# Autodesk Inventor assembly: Kippschalter
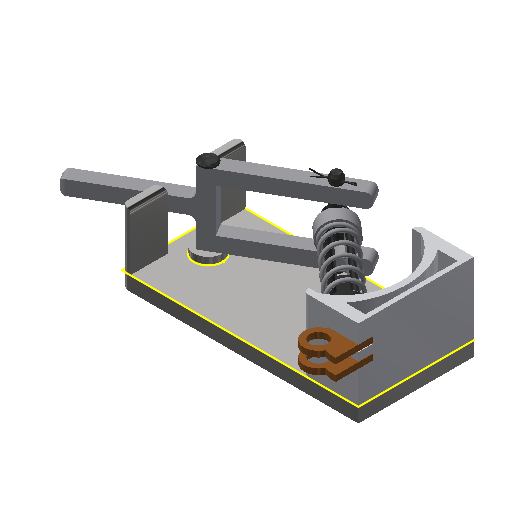
[picture p0: Inventor's stored thumbnail of the model, 512x512]
Saved by Autodesk Inventor 2025.3 (Build 293356000, 356)
## iProperties
Created: 2025-01-24
Part Number: Kippschalter
Material: Generisch
Document SubType Name: Assembly
Designer: abdel
Author: abdel
## Documents named in this file (12)
- C:\Users\abdel\Documents\Inventor\Projektname\Beleg Me2\Kippschalter.iam
- C:\Users\abdel\Documents\Inventor\Projektname\Beleg Me2\Feder.ipt
- C:\Users\abdel\Documents\Inventor\Projektname\Beleg Me2\Federbalken.ipt
- C:\Users\abdel\Documents\Inventor\Projektname\Beleg Me2\Federteller.ipt
- C:\Users\abdel\Documents\Inventor\Projektname\Beleg Me2\Hebel.ipt
- C:\Users\abdel\Documents\Inventor\Projektname\Beleg Me2\Leistende Kontakt.ipt
- C:\Users\abdel\Documents\Inventor\Projektname\Beleg Me2\Gehäuse.ipt
- C:\Users\abdel\Documents\Inventor\Projektname\Beleg Me2\Gehäuse_Kurve .ipt
- C:\Users\abdel\Documents\Inventor\Projektname\Beleg Me2\Kontakt.ipt
- C:\Users\abdel\Documents\Inventor\Content Center Files\R2025\de-DE\ISO 2341(2)\ISO 2341 - B - 4 x 35DIN EN.ipt
- C:\Users\abdel\Documents\Inventor\Content Center Files\R2025\de-DE\ISO 2341(2)\ISO 2341 - B - 4 x 28DIN EN.ipt
- C:\Users\abdel\Documents\Inventor\Content Center Files\R2025\de-DE\ISO 1234(2)\ISO 1234 - 0,6 x 10ISO.ipt
## Components (13 placed, 11 different names)
1. Gehäuse:1 — Drehbar:4, Starr:8, Passend:11, Passend:12
2. Feder:1 — Passend:1, Passend:2, Fluchtend:1
3. Federbalken:1 — Passend:1, Passend:2, Passend:3, Starr:2
4. Federteller:1 — Passend:3, Fluchtend:1
5. Hebel:1 — Drehbar:4, Passend:16, Passend:17, Passend:18, Passend:19
6. Leistende Kontakt:1 — Starr:2, Passend:4, Passend:5, Passend:14
7. Gehäuse_Kurve :1 — Starr:8, Fluchtend:2, Passend:15
8. Kontakt:3 — Passend:4, Passend:5
9. Kontakt:4 — Passend:14, Passend:15
10. DIN EN 22341 B B - 4 x 35:1 — Passend:16, Passend:17, Starr:10
11. DIN EN 22341 B B - 4 x 28:1 — Passend:18, Passend:19, Starr:9
12. ISO 1234 0,6 x 10:1 — Starr:9
13. ISO 1234 0,6 x 10:2 — Starr:10
## Relationships (20: Mate 13, WeldJoint 4, Flush 2, RevoluteJoint 1)
- Passend:1 [Mate]: Feder:1 ↔ Federbalken:1
- Passend:2 [Mate]: Feder:1 ↔ Federbalken:1
- Passend:3 [Mate]: Federbalken:1 ↔ Federteller:1
- Fluchtend:1 [Flush]: Feder:1 ↔ Federteller:1
- Starr:2 [WeldJoint]: Federbalken:1 ↔ Leistende Kontakt:1
- Passend:4 [Mate]: Leistende Kontakt:1 ↔ Kontakt:3
- Passend:5 [Mate]: Leistende Kontakt:1 ↔ Kontakt:3
- Drehbar:4 [RevoluteJoint]: Gehäuse:1 ↔ Hebel:1
- Starr:8 [WeldJoint]: Gehäuse:1 ↔ Gehäuse_Kurve :1
- Fluchtend:2 [Flush]: Gehäuse_Kurve :1
- Passend:11 [Mate]: Gehäuse:1
- Passend:12 [Mate]: Gehäuse:1
- Passend:14 [Mate]: Leistende Kontakt:1 ↔ Kontakt:4
- Passend:15 [Mate]: Gehäuse_Kurve :1 ↔ Kontakt:4
- Passend:16 [Mate]: Hebel:1 ↔ DIN EN 22341 B B - 4 x 35:1
- Passend:17 [Mate]: Hebel:1 ↔ DIN EN 22341 B B - 4 x 35:1
- Passend:18 [Mate]: Hebel:1 ↔ DIN EN 22341 B B - 4 x 28:1
- Passend:19 [Mate]: Hebel:1 ↔ DIN EN 22341 B B - 4 x 28:1
- Starr:9 [WeldJoint]: DIN EN 22341 B B - 4 x 28:1 ↔ ISO 1234 0,6 x 10:1
- Starr:10 [WeldJoint]: DIN EN 22341 B B - 4 x 35:1 ↔ ISO 1234 0,6 x 10:2
